# Autodesk Inventor assembly: mini Cryostat
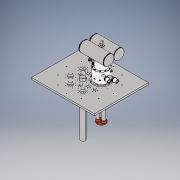
[picture p0: Inventor's stored thumbnail of the model, 180x180]
Saved by Autodesk Inventor 2018 (Build 220112000, 112)
## iProperties
Created: 2018-10-10
Part Number: mini Cryostat
Document SubType Name: Assembly
Designer: Admin
Author: Admin
## Documents named in this file (9)
- C:\Users\freyja\Documents\Cryorefrigerator\CAD\mini Cryostat.iam
- C:\Users\freyja\Documents\Cryorefrigerator\CAD\External Models\CH40415 24JUL14 C.ipt
- C:\Users\freyja\Documents\Cryorefrigerator\CAD\vacuum jacket long.ipt
- C:\Users\freyja\Documents\Cryorefrigerator\CAD\vacuum jacket.ipt
- C:\Users\freyja\Documents\Cryorefrigerator\CAD\Top Plate V2.2.ipt
- C:\Users\freyja\Documents\Cryorefrigerator\CAD\foot type 1.iam
- C:\Users\freyja\Documents\Cryorefrigerator\CAD\mini 55K stage.ipt
- C:\Users\freyja\Documents\Cryorefrigerator\CAD\still pipe standin.ipt
- C:\Users\freyja\Documents\Cryorefrigerator\CAD\foot type 2.iam
## Components (16 placed, 8 different names)
1. Top Plate V2.2:1 — Mate:16, Mate:18, Mate:19, Mate:20, Mate:21, Mate:26, Mate:37, Mate:38, Mate:39, Mate:40, Mate:41, Mate:42, Mate:43, Mate:44, Mate:47, Mate:49, Mate:50, Mate:51, Mate:52, Mate:53, Mate:54, Mate:55, Mate:56, Mate:57, Mate:58, Mate:59, Mate:60
2. CH40415 24JUL14 C:1 — Mate:16, Mate:18, Mate:26, Mate:46, Flush:1
3. vacuum jacket long:1 — Mate:7, Mate:8, Mate:9
4. vacuum jacket:1 — Mate:7, Mate:8, Mate:9, Mate:19, Mate:20, Mate:21
5. foot type 1:1 [sub-assembly] — Mate:37, Mate:43
6. foot type 1:2 [sub-assembly] — Mate:40, Mate:41
7. foot type 1:3 [sub-assembly] — Mate:39, Mate:42
8. foot type 1:4 [sub-assembly] — Mate:38, Mate:44
9. mini 55K stage:1 — Mate:46, Mate:48, Flush:1
10. still pipe standin:1 — Mate:47, Mate:48
11. foot type 2:1 [sub-assembly] — Mate:49, Mate:50
12. foot type 2:2 [sub-assembly] — Mate:51, Mate:56
13. foot type 2:3 [sub-assembly] — Mate:53, Mate:54
14. foot type 2:4 [sub-assembly] — Mate:52, Mate:55
15. foot type 2:5 [sub-assembly] — Mate:57, Mate:60
16. foot type 2:6 [sub-assembly] — Mate:58, Mate:59
## Relationships (33: Mate 32, Flush 1)
- Mate:7: vacuum jacket long:1 ↔ vacuum jacket:1
- Mate:8: vacuum jacket long:1 ↔ vacuum jacket:1
- Mate:9: vacuum jacket long:1 ↔ vacuum jacket:1
- Mate:16: Top Plate V2.2:1 ↔ CH40415 24JUL14 C:1
- Mate:18: Top Plate V2.2:1 ↔ CH40415 24JUL14 C:1
- Mate:19: Top Plate V2.2:1 ↔ vacuum jacket:1
- Mate:20: Top Plate V2.2:1 ↔ vacuum jacket:1
- Mate:21: Top Plate V2.2:1 ↔ vacuum jacket:1
- Mate:26: Top Plate V2.2:1 ↔ CH40415 24JUL14 C:1
- Mate:37: Top Plate V2.2:1 ↔ foot type 1:1
- Mate:38: Top Plate V2.2:1 ↔ foot type 1:4
- Mate:39: Top Plate V2.2:1 ↔ foot type 1:3
- Mate:40: Top Plate V2.2:1 ↔ foot type 1:2
- Mate:41: Top Plate V2.2:1 ↔ foot type 1:2
- Mate:42: Top Plate V2.2:1 ↔ foot type 1:3
- Mate:43: Top Plate V2.2:1 ↔ foot type 1:1
- Mate:44: Top Plate V2.2:1 ↔ foot type 1:4
- Mate:46: CH40415 24JUL14 C:1 ↔ mini 55K stage:1
- Mate:47: Top Plate V2.2:1 ↔ still pipe standin:1
- Mate:48: mini 55K stage:1 ↔ still pipe standin:1
- Flush:1: CH40415 24JUL14 C:1 ↔ mini 55K stage:1
- Mate:49: Top Plate V2.2:1 ↔ foot type 2:1
- Mate:50: Top Plate V2.2:1 ↔ foot type 2:1
- Mate:51: Top Plate V2.2:1 ↔ foot type 2:2
- Mate:52: Top Plate V2.2:1 ↔ foot type 2:4
- Mate:53: Top Plate V2.2:1 ↔ foot type 2:3
- Mate:54: Top Plate V2.2:1 ↔ foot type 2:3
- Mate:55: Top Plate V2.2:1 ↔ foot type 2:4
- Mate:56: Top Plate V2.2:1 ↔ foot type 2:2
- Mate:57: Top Plate V2.2:1 ↔ foot type 2:5
- Mate:58: Top Plate V2.2:1 ↔ foot type 2:6
- Mate:59: Top Plate V2.2:1 ↔ foot type 2:6
- Mate:60: Top Plate V2.2:1 ↔ foot type 2:5
